# Autodesk Inventor assembly: 2018 radiator analysis
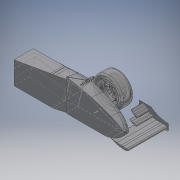
[picture p0: Inventor's stored thumbnail of the model, 180x180]
Saved by Autodesk Inventor 2018.2 (Build 222227000, 227)
## iProperties
Company: none
Created: 2018-02-25
Part Number: 2018 radiator analysis
Material: 一般
Description: CATIA V5 STEP Exchange
Document SubType Name: Assembly
Designer: ku_sk
Authority: none
Sending System: CATIA V5 STEP AP203
Preprocessor: CATIA Version 5 Release 17 (IN-10)
Title: Z:\各班フォルダ\2018\ボディ\カウル\AeroCAD2018\設計\2018 radiator analysis.stp
Author: none
## Documents named in this file (5)
- C:\Users\ku_sk\Documents\Inventor\AeroCAD2018\設計\Fr.wing\2018 radiator analysis.iam
- C:\Users\ku_sk\Documents\Inventor\AeroCAD2018\設計\Fr.wing\body\AssyTsutsui2018.iam
- C:\Users\ku_sk\Documents\Inventor\AeroCAD2018\設計\Fr.wing\body\SidePanel_Upper.ipt
- C:\Users\ku_sk\Documents\Inventor\AeroCAD2018\設計\Fr.wing\body\aaa.ipt
- C:\Users\ku_sk\Documents\Inventor\AeroCAD2018\設計\Fr.wing\Fr.wing.iam
## Components (4 placed, 4 different names)
1. AssyTsutsui2018.1 [sub-assembly]
2. Part127.1
3. 2018Frontnose — フラッシュ:1
4. Fr.wing:1 [sub-assembly] — フラッシュ:1
## Relationships (1: Flush 1)
- フラッシュ:1 [Flush]: 2018Frontnose ↔ Fr.wing:1
